# Autodesk Inventor assembly: Assembly1
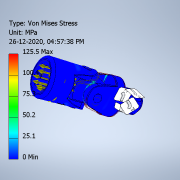
[picture p0: Inventor's stored thumbnail of the model, 180x180]
Saved by Autodesk Inventor 2020 (Build 240168000, 168)
## iProperties
Created: 2020-12-25
Part Number: Assembly1
Document SubType Name: Assembly
Designer: Vikki
Author: Vikki
## Documents named in this file (10)
- D:\borewell rescuebot\pll manipulator files\sps manipulator\Assembly1.iam
- D:\borewell rescuebot\pll manipulator files\sps manipulator\craftsman-3-pc-universal-joint-set-1.snapshot.1\Craftsman Socket U-Joint Drive.ipt
- D:\borewell rescuebot\pll manipulator files\sps manipulator\craftsman-3-pc-universal-joint-set-1.snapshot.1\Craftsman Socket U-Joint Intermediate Body.ipt
- D:\borewell rescuebot\pll manipulator files\sps manipulator\craftsman-3-pc-universal-joint-set-1.snapshot.1\Craftsman Socket U-Joint Base.ipt
- D:\borewell rescuebot\pll manipulator files\sps manipulator\Assembly1\AIP\FEA\dgr59qlsw.fins
- D:\borewell rescuebot\pll manipulator files\sps manipulator\Assembly1\AIP\FEA\dgr59qlsw.fsat
- D:\borewell rescuebot\pll manipulator files\sps manipulator\Assembly1\AIP\FEA\dgr59qlsw.ftes
- D:\borewell rescuebot\pll manipulator files\sps manipulator\Assembly1\AIP\FEA\dgr59qlsw.fwiz
- D:\borewell rescuebot\pll manipulator files\sps manipulator\Assembly1\AIP\FEA\dgr59qlts.fmsh
- D:\borewell rescuebot\pll manipulator files\sps manipulator\Assembly1\AIP\FEA\dgr59qltt.fres
## Components (3 placed, 3 different names)
1. Craftsman Socket U-Joint Drive:1 — Mate:1, Mate:4
2. Craftsman Socket U-Joint Intermediate Body:1 — Mate:1, Mate:3
3. Craftsman Socket U-Joint Base:1 — Mate:3, Mate:4
## Relationships (3: Mate 3)
- Mate:1: Craftsman Socket U-Joint Drive:1 ↔ Craftsman Socket U-Joint Intermediate Body:1
- Mate:3: Craftsman Socket U-Joint Intermediate Body:1 ↔ Craftsman Socket U-Joint Base:1
- Mate:4: Craftsman Socket U-Joint Drive:1 ↔ Craftsman Socket U-Joint Base:1
## Named parameters: sa_0 = 14700, sa_1 = 20000
note: some values were not read from the file. Shown as the stored number, unit unknown: "sa_0", "sa_1".
